# Autodesk Inventor assembly: body_1
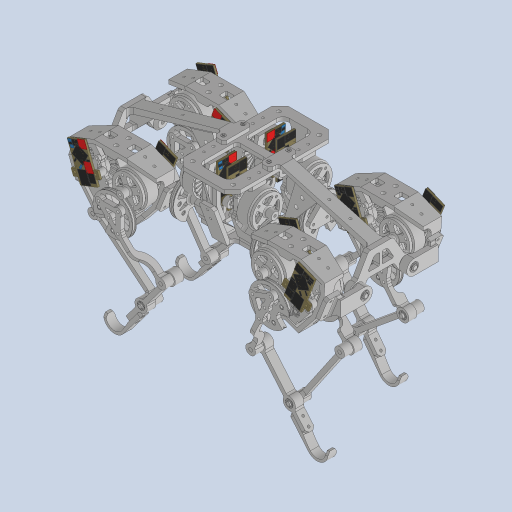
[picture p0: Inventor's stored thumbnail of the model, 512x512]
Saved by Autodesk Inventor 2023 (Build 270158000, 158)
## iProperties
Created: 2020-12-19
Part Number: body_1
Document SubType Name: Assembly
Designer: Shuang Peng
Author: Shuang Peng
## Documents named in this file (11)
- D:\projects-3\biped_tiny\hardware\body_1.iam
- D:\projects-3\biped_tiny\hardware\leg_1.iam
- D:\projects-3\biped_tiny\hardware\leg_1_MIR.iam
- D:\projects-3\biped_tiny\hardware\body_conn_2.ipt
- D:\projects-3\biped_tiny\hardware\body_shell_1.ipt
- D:\projects-3\biped_tiny\hardware\body_shell_2.ipt
- D:\projects-3\biped_tiny\hardware\body_conn_2_MIR.ipt
- D:\projects-3\biped_tiny\hardware\fr_bearing_s_1.ipt
- D:\projects-3\biped_tiny\hardware\bearing_3_6_2.ipt
- D:\projects-3\biped_tiny\hardware\pin_3_10.ipt
- D:\projects-3\biped_tiny\hardware\screw_2_4.ipt
## Components (24 placed, 10 different names)
1. leg_1:1 [sub-assembly] — Flush:2, Flush:3, Mate:2, Flush:4, Flush:8, Mate:3, Flush:9, Flush:10, Flush:11, Insert:1, Insert:2, Insert:5, Insert:7, Insert:8
2. leg_1_MIR:1 [sub-assembly] — Flush:2, Flush:3, Mate:2, Flush:5, Insert:3, Insert:4
3. leg_1:2 [sub-assembly] — Flush:4, Flush:5, Flush:6, Flush:7, Insert:11, Insert:12
4. leg_1_MIR:2 [sub-assembly] — Flush:6, Flush:7, Flush:8, Mate:3, Insert:6, Insert:13, Insert:14
5. body_conn_2:1 — Flush:9, Insert:1, Insert:2, Flush:12, Insert:17
6. body_shell_1:1 — Flush:10, Insert:5, Insert:6, Insert:9, Insert:10, Insert:15, Insert:16, Flush:13
7. body_shell_2:1 — Flush:11, Insert:7, Insert:8, Mate:4
8. body_conn_2_MIR:1 — Insert:3, Insert:4, Insert:18
9. fr_bearing_s_1:1 — Flush:12, Insert:9, Insert:10, Insert:25, Insert:26
10. body_conn_2:2 — Insert:11, Insert:12, Insert:20
11. body_conn_2_MIR:2 — Insert:13, Insert:14, Insert:19
12. fr_bearing_s_1:2 — Insert:15, Insert:16, Insert:27, Insert:28
13. bearing_3_6_2:1 — Insert:17, Insert:21
14. bearing_3_6_2:2 — Insert:18, Insert:22
15. bearing_3_6_2:3 — Insert:19, Insert:23
16. bearing_3_6_2:4 — Insert:20, Insert:24
17. pin_3_10:1 — Insert:21
18. pin_3_10:2 — Insert:22
19. pin_3_10:3 — Insert:24
20. pin_3_10:4 — Insert:23
21. screw_2_4:1 — Insert:28
22. screw_2_4:2 — Insert:27
23. screw_2_4:3 — Insert:25
24. screw_2_4:4 — Insert:26
## Relationships (43: Insert 28, Flush 12, Mate 3)
- Flush:2: leg_1:1 ↔ leg_1_MIR:1
- Flush:3: leg_1:1 ↔ leg_1_MIR:1
- Mate:2 (25 mm): leg_1:1 ↔ leg_1_MIR:1
- Flush:4: leg_1:1 ↔ leg_1:2
- Flush:5: leg_1_MIR:1 ↔ leg_1:2
- Flush:6: leg_1:2 ↔ leg_1_MIR:2
- Flush:7: leg_1:2 ↔ leg_1_MIR:2
- Flush:8: leg_1:1 ↔ leg_1_MIR:2
- Mate:3 (20 mm): leg_1:1 ↔ leg_1_MIR:2
- Flush:9: leg_1:1 ↔ body_conn_2:1
- Flush:10: leg_1:1 ↔ body_shell_1:1
- Flush:11: leg_1:1 ↔ body_shell_2:1
- Insert:1: leg_1:1 ↔ body_conn_2:1
- Insert:2: leg_1:1 ↔ body_conn_2:1
- Insert:3: leg_1_MIR:1 ↔ body_conn_2_MIR:1
- Insert:4: leg_1_MIR:1 ↔ body_conn_2_MIR:1
- Flush:12: body_conn_2:1 ↔ fr_bearing_s_1:1
- Insert:5: leg_1:1 ↔ body_shell_1:1
- Insert:6: leg_1_MIR:2 ↔ body_shell_1:1
- Insert:7: leg_1:1 ↔ body_shell_2:1
- Insert:8: leg_1:1 ↔ body_shell_2:1
- Insert:9: body_shell_1:1 ↔ fr_bearing_s_1:1
- Insert:10: body_shell_1:1 ↔ fr_bearing_s_1:1
- Insert:11: leg_1:2 ↔ body_conn_2:2
- Insert:12: leg_1:2 ↔ body_conn_2:2
- Insert:13: leg_1_MIR:2 ↔ body_conn_2_MIR:2
- Insert:14: leg_1_MIR:2 ↔ body_conn_2_MIR:2
- Insert:15: body_shell_1:1 ↔ fr_bearing_s_1:2
- Insert:16: body_shell_1:1 ↔ fr_bearing_s_1:2
- Insert:17: body_conn_2:1 ↔ bearing_3_6_2:1
- Insert:18: body_conn_2_MIR:1 ↔ bearing_3_6_2:2
- Insert:19: body_conn_2_MIR:2 ↔ bearing_3_6_2:3
- Insert:20: body_conn_2:2 ↔ bearing_3_6_2:4
- Insert:21 (-1 mm): bearing_3_6_2:1 ↔ pin_3_10:1
- Insert:22 (-1 mm): bearing_3_6_2:2 ↔ pin_3_10:2
- Insert:23 (-1 mm): bearing_3_6_2:3 ↔ pin_3_10:4
- Insert:24 (-1 mm): bearing_3_6_2:4 ↔ pin_3_10:3
- Insert:25: fr_bearing_s_1:1 ↔ screw_2_4:3
- Insert:26: fr_bearing_s_1:1 ↔ screw_2_4:4
- Insert:27: fr_bearing_s_1:2 ↔ screw_2_4:2
- Insert:28: fr_bearing_s_1:2 ↔ screw_2_4:1
- Mate:4: body_shell_2:1
- Flush:13: body_shell_1:1
